# Autodesk Inventor assembly: M - Climber Upper Rails
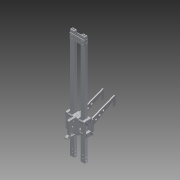
[picture p0: Inventor's stored thumbnail of the model, 180x180]
Saved by Autodesk Inventor 2013 (Build 170138000, 138)
## iProperties
Created: 2013-02-17
Part Number: M - Climber Upper Rails
Document SubType Name: Assembly
Designer: Moses
Mass: 3225.79 g
Surface Area: 4928.67 cm^2
Volume: 752.838 cm^3
Density: 4.28484 g/cm^3
Author: Moses
## Documents named in this file (6)
- C:\Users\Arpan\Documents\GitHub\frc2013CAD\M-Climber\M - Climber Upper Rails.iam
- C:\Users\Arpan\Documents\GitHub\frc2013CAD\M-Climber\M - Rail 1.iam
- C:\Users\Arpan\Documents\GitHub\frc2013CAD\M-Climber\M - hook block.iam
- C:\Users\Arpan\Documents\GitHub\frc2013CAD\M-Climber\M - Carriage.iam
- C:\Users\Arpan\Documents\GitHub\frc2013CAD\M-Climber\M - Upper Rail Connector Plate 1.ipt
- C:\Users\Arpan\Documents\GitHub\frc2013CAD\M-Climber\91257A560\91257A560.ipt
## Components (9 placed, 5 different names)
1. M - Rail 1:1 [sub-assembly] — Flush:1, Flush:2, Mate:1, Tangent:1, Mate:3, Tangent:2, Mate:5, Mate:7, Mate:8, Mate:9
2. M - Rail 1:2 [sub-assembly] — Flush:1, Flush:2, Mate:1, Mate:2, Mate:4, Tangent:3, Tangent:4, Mate:6, Mate:10, Flush:6
3. M - hook block:1 [sub-assembly] — Mate:2, Flush:4, Flush:5
4. M - Carriage:1 [sub-assembly] — Tangent:1, Mate:3, Tangent:2, Flush:3, Insert:1, Insert:2
5. M - Carriage:2 [sub-assembly] — Mate:4, Tangent:3, Tangent:4, Flush:3, Flush:4, Flush:5, Flush:6
6. M - Upper Rail Connector Plate 1:1 — Mate:5, Mate:6, Mate:7
7. M - Upper Rail Connector Plate 1:2 — Mate:8, Mate:9, Mate:10
8. 91257A560:1 — Insert:2
9. 91257A560:2 — Insert:1
## Relationships (22: Mate 10, Flush 6, Tangent 4, Insert 2)
- Flush:1: M - Rail 1:1 ↔ M - Rail 1:2
- Flush:2: M - Rail 1:1 ↔ M - Rail 1:2
- Mate:1 (38.1 mm): M - Rail 1:1 ↔ M - Rail 1:2
- Mate:2 (12.7 mm): M - Rail 1:2 ↔ M - hook block:1
- Tangent:1: M - Rail 1:1 ↔ M - Carriage:1
- Mate:3: M - Rail 1:1 ↔ M - Carriage:1
- Tangent:2: M - Rail 1:1 ↔ M - Carriage:1
- Mate:4: M - Rail 1:2 ↔ M - Carriage:2
- Tangent:3: M - Rail 1:2 ↔ M - Carriage:2
- Tangent:4: M - Rail 1:2 ↔ M - Carriage:2
- Flush:3: M - Carriage:1 ↔ M - Carriage:2
- Flush:4: M - hook block:1 ↔ M - Carriage:2
- Flush:5 (-41.275 mm): M - hook block:1 ↔ M - Carriage:2
- Mate:5: M - Rail 1:1 ↔ M - Upper Rail Connector Plate 1:1
- Mate:6: M - Rail 1:2 ↔ M - Upper Rail Connector Plate 1:1
- Mate:7: M - Rail 1:1 ↔ M - Upper Rail Connector Plate 1:1
- Mate:8: M - Rail 1:1 ↔ M - Upper Rail Connector Plate 1:2
- Mate:9: M - Rail 1:1 ↔ M - Upper Rail Connector Plate 1:2
- Mate:10: M - Rail 1:2 ↔ M - Upper Rail Connector Plate 1:2
- Insert:1: M - Carriage:1 ↔ 91257A560:2
- Insert:2: M - Carriage:1 ↔ 91257A560:1
- Flush:6 (139.7 mm): M - Rail 1:2 ↔ M - Carriage:2
